# Autodesk Inventor assembly: pot1_assy
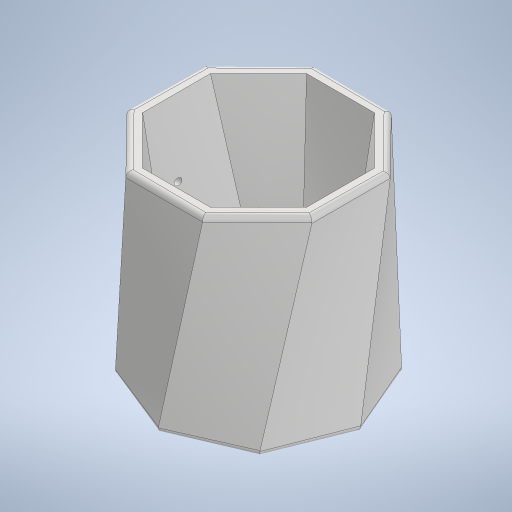
[picture p0: Inventor's stored thumbnail of the model, 512x512]
Saved by Autodesk Inventor 2023 (Build 270158000, 158)
## iProperties
Created: 2025-10-09
Part Number: pot1_assy
Document SubType Name: Assembly
Designer: Justin Pascual
Author: Justin Pascual
## Documents named in this file (3)
- C:\Users\Justin Pascual\Documents\GitHub\modular-flower-pot\pot1_assy.iam
- C:\Users\Justin Pascual\Documents\GitHub\modular-flower-pot\pot1.ipt
- C:\Users\Justin Pascual\Documents\GitHub\modular-flower-pot\dovetail.ipt
## Components (2 placed, 2 different names)
1. pot1:1 — Mate:1, Flush:1, Flush:2
2. dovetail:1 — Mate:1, Flush:1, Flush:2
## Relationships (3: Flush 2, Mate 1)
- Mate:1: pot1:1 ↔ dovetail:1
- Flush:1: pot1:1 ↔ dovetail:1
- Flush:2: pot1:1 ↔ dovetail:1
